# Autodesk Inventor assembly: Assembly1
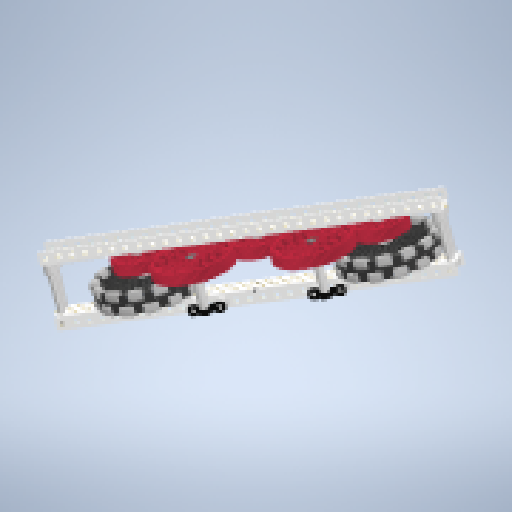
[picture p0: Inventor's stored thumbnail of the model, 512x512]
Saved by Autodesk Inventor 2024 (Build 280153000, 153)
## iProperties
Created: 2023-09-19
Part Number: Assembly1
Document SubType Name: Assembly
Designer: Robodox
Author: Robodox
## Documents named in this file (18)
- C:\Users\Robodox\Documents\GitHub\VEXCAD\Assembly1.iam
- C:\Users\Robodox\Documents\GitHub\VEX-CAD-Inventor\Structure\C Channel\Aluminum 1x2x1\Alu C 1x2x1x30.ipt
- C:\Users\Robodox\Documents\GitHub\VEX-CAD-Inventor\Motion\Gears\HS Gear.iam
- C:\Users\Robodox\Documents\GitHub\VEXCAD\Part1.ipt
- C:\Users\Robodox\Documents\GitHub\VEXCAD\Part2.ipt
- C:\Users\Robodox\Documents\GitHub\VEXCAD\Part3.ipt
- C:\Users\Robodox\Documents\GitHub\VEX-CAD-Inventor\Motion\Spacers\Washer Steel\SWasher .375 OD x .031250.ipt
- C:\Users\Robodox\Documents\GitHub\VEX-CAD-Inventor\Motion\Spacers\Washer Steel.ipt
- C:\Users\Robodox\Documents\GitHub\VEXCAD\Part4.ipt
- C:\Users\Robodox\Downloads\2020 VRC Library-BNS-SID-YY-EZ\2020 BNS-VRC-SID-YY Library\Motion\Pillow Bearing Block.ipt
- C:\Users\Robodox\Documents\GitHub\VEXCAD\Part5.ipt
- C:\Users\Robodox\Downloads\2020 VRC Library-BNS-SID-YY-EZ\2020 BNS-VRC-SID-YY Library\Motion\Bearing Flat.ipt
- C:\Users\Robodox\Documents\GitHub\VEXCAD\part8.ipt
- C:\Users\Robodox\Downloads\2020 VRC Library-BNS-SID-YY-EZ\2020 BNS-VRC-SID-YY Library\Motion\Shaft Collar.ipt
- C:\Users\Robodox\Documents\GitHub\VEX-CAD-Inventor\Motion\Wheels\Omni Wheel\4 Omni AS, Square.iam
- C:\Users\Robodox\Documents\GitHub\VEX-CAD-Inventor\Motion\Wheels\Omni Wheel.iam
- C:\Users\Robodox\Documents\GitHub\VEX-CAD-Inventor\Motion\Gears\HS Gear\HS 72T Gear, Square.iam
- C:\Users\Robodox\Documents\GitHub\VEX-CAD-Inventor\Motion\Gears\HS Gear\HS 48T Gear, Square.iam
## Components (61 placed, 14 different names)
1. Alu C 1x2x1x30:1 — Flush:1, Flush:2, Mate:1, Mate:2, Mate:7, Mate:11, Mate:12, Mate:15, Mate:17, Mate:19, Mate:27, Mate:31, Mate:32, Mate:33, Mate:34, Mate:35, Mate:36, Mate:37, Mate:38, Mate:56, Mate:57, Mate:58, Mate:59, Mate:60, Mate:61, Mate:62, Mate:63, Mate:64
2. Alu C 1x2x1x30:2 — Flush:1, Flush:2, Mate:20, Mate:21, Mate:68, Mate:71, Mate:74
3. Part2:5 — Mate:13, Mate:14, Mate:28, Mate:29
4. Part1:9 — Mate:14, Mate:29
5. Part1:10 — Mate:12, Mate:13, Mate:15, Mate:28
6. Part3:3 — Mate:31, Mate:32, Mate:39, Mate:40
7. Part3:4 — Mate:33, Mate:38, Mate:41
8. Part3:5 — Mate:34, Mate:37, Mate:42, Mate:43
9. Part3:6 — Mate:35, Mate:36, Mate:44
10. Pillow Bearing Block:1 — Mate:39, Mate:40, Mate:41, Mate:50, Mate:51
11. Pillow Bearing Block:2 — Mate:42, Mate:43, Mate:44, Mate:46, Mate:53
12. Part5:1 — Mate:47, Mate:52, Mate:94, Mate:96
13. Part5:2 — Mate:48, Mate:49, Mate:95, Mate:97
14. Part5:3 — Mate:46, Mate:47, Mate:52, Mate:53
15. Part5:4 — Mate:48, Mate:49, Mate:50, Mate:51
16. Bearing Flat:1 — Mate:56, Mate:59, Mate:60, Mate:72, Mate:86, Mate:88
17. Bearing Flat:2 — Mate:57, Mate:61, Mate:62, Mate:75
18. Bearing Flat:3 — Mate:58, Mate:63, Mate:64, Mate:69, Mate:91
19. part8:1 — Mate:68, Mate:69, Mate:98, Mate:99
20. part8:2 — Mate:71, Mate:72, Mate:106, Mate:107
21. part8:3 — Mate:74, Mate:75, Mate:102, Mate:103
22. Part3:11 — Mate:90
23. Part3:12 — Mate:87, Mate:100, Mate:101
24. Shaft Collar:1 — Mate:86, Mate:89, Mate:104, Mate:105
25. Shaft Collar:2 — Mate:92, Mate:93
26. 4 Omni AS, Square:1 [sub-assembly] — Mate:87, Mate:88, Mate:89
27. 4 Omni AS, Square:2 [sub-assembly] — Mate:90, Mate:91, Mate:92, Mate:93
28. HS 72T Gear, Square:8 [sub-assembly] — Mate:94, Mate:96
29. HS 72T Gear, Square:9 [sub-assembly] — Mate:95, Mate:97
30. HS 48T Gear, Square:10 [sub-assembly] — Mate:98, Mate:99
31. HS 48T Gear, Square:11 [sub-assembly] — Mate:100, Mate:101, Mate:106, Mate:107
32. HS 48T Gear, Square:12 [sub-assembly] — Mate:102, Mate:103
33. SWasher .375 OD x .031250:5 — Mate:104, Mate:105
34. Part1:1 — Mate:4, Mate:5
35. Part2:1 — Mate:3, Mate:4, Mate:5, Mate:6
36. Part1:2 — Mate:1, Mate:2, Mate:3, Mate:6
37. Part1:3
38. Part2:2
39. Part1:4
40. Part1:6 — Mate:9, Mate:10
41. Part2:3 — Mate:8, Mate:9, Mate:10, Mate:30
42. Part1:5 — Mate:7, Mate:8, Mate:11, Mate:30
43. Part1:7
44. Part2:4
45. Part1:8
46. Part1:11 — Mate:16, Mate:17, Mate:18, Mate:19, Mate:26
47. Part2:6 — Mate:16, Mate:18
48. Part1:12
49. Part2:7
50. Part3:1 — Mate:20, Mate:21, Mate:22, Mate:23, Mate:25
51. Part4:1 — Mate:24, Mate:25, Mate:26, Mate:27
52. SWasher .375 OD x .031250:1 — Mate:22, Mate:23, Mate:24
53. Part3:2
54. Part4:2
55. SWasher .375 OD x .031250:2
56. Part3:8
57. Part4:3
58. SWasher .375 OD x .031250:3
59. Part3:9
60. Part4:4
61. SWasher .375 OD x .031250:4
## Component patterns: (2 elements, first: Part1:1 + Part2:1 + Part1:2), (2 elements, first: Part1:6 + Part2:3 + Part1:5), (2 elements, first: Part1:11 + Part2:6), (2 elements), (2 elements, first: Part3:1 + Part4:1 + SWasher .375 OD x .031250:1), Component Pattern 4:2 (2 elements)
## Relationships (91: Mate 89, Flush 2)
- Flush:1: Alu C 1x2x1x30:1 ↔ Alu C 1x2x1x30:2
- Flush:2: Alu C 1x2x1x30:1 ↔ Alu C 1x2x1x30:2
- Mate:1: Alu C 1x2x1x30:1 ↔ Part1:2
- Mate:2: Alu C 1x2x1x30:1 ↔ Part1:2
- Mate:3: Part2:1 ↔ Part1:2
- Mate:4: Part1:1 ↔ Part2:1
- Mate:5: Part1:1 ↔ Part2:1
- Mate:6: Part2:1 ↔ Part1:2
- Mate:7: Alu C 1x2x1x30:1 ↔ Part1:5
- Mate:8: Part2:3 ↔ Part1:5
- Mate:9: Part1:6 ↔ Part2:3
- Mate:10: Part1:6 ↔ Part2:3
- Mate:11: Alu C 1x2x1x30:1 ↔ Part1:5
- Mate:12: Alu C 1x2x1x30:1 ↔ Part1:10
- Mate:13: Part2:5 ↔ Part1:10
- Mate:14: Part2:5 ↔ Part1:9
- Mate:15: Alu C 1x2x1x30:1 ↔ Part1:10
- Mate:16: Part1:11 ↔ Part2:6
- Mate:17: Alu C 1x2x1x30:1 ↔ Part1:11
- Mate:18: Part1:11 ↔ Part2:6
- Mate:19: Alu C 1x2x1x30:1 ↔ Part1:11
- Mate:20: Alu C 1x2x1x30:2 ↔ Part3:1
- Mate:21: Alu C 1x2x1x30:2 ↔ Part3:1
- Mate:22: Part3:1 ↔ SWasher .375 OD x .031250:1
- Mate:23: Part3:1 ↔ SWasher .375 OD x .031250:1
- Mate:24: Part4:1 ↔ SWasher .375 OD x .031250:1
- Mate:25: Part3:1 ↔ Part4:1
- Mate:26: Part1:11 ↔ Part4:1
- Mate:27: Alu C 1x2x1x30:1 ↔ Part4:1
- Mate:28: Part2:5 ↔ Part1:10
- Mate:29: Part2:5 ↔ Part1:9
- Mate:30: Part2:3 ↔ Part1:5
- Mate:31: Alu C 1x2x1x30:1 ↔ Part3:3
- Mate:32: Alu C 1x2x1x30:1 ↔ Part3:3
- Mate:33: Alu C 1x2x1x30:1 ↔ Part3:4
- Mate:34: Alu C 1x2x1x30:1 ↔ Part3:5
- Mate:35: Alu C 1x2x1x30:1 ↔ Part3:6
- Mate:36: Alu C 1x2x1x30:1 ↔ Part3:6
- Mate:37: Alu C 1x2x1x30:1 ↔ Part3:5
- Mate:38: Alu C 1x2x1x30:1 ↔ Part3:4
- Mate:39: Part3:3 ↔ Pillow Bearing Block:1
- Mate:40: Part3:3 ↔ Pillow Bearing Block:1
- Mate:41: Part3:4 ↔ Pillow Bearing Block:1
- Mate:42: Part3:5 ↔ Pillow Bearing Block:2
- Mate:43: Part3:5 ↔ Pillow Bearing Block:2
- Mate:44: Part3:6 ↔ Pillow Bearing Block:2
- Mate:46: Pillow Bearing Block:2 ↔ Part5:3
- Mate:47: Part5:1 ↔ Part5:3
- Mate:48: Part5:2 ↔ Part5:4
- Mate:49: Part5:2 ↔ Part5:4
- Mate:50: Pillow Bearing Block:1 ↔ Part5:4
- Mate:51: Pillow Bearing Block:1 ↔ Part5:4
- Mate:52: Part5:1 ↔ Part5:3
- Mate:53: Pillow Bearing Block:2 ↔ Part5:3
- Mate:56: Alu C 1x2x1x30:1 ↔ Bearing Flat:1
- Mate:57: Alu C 1x2x1x30:1 ↔ Bearing Flat:2
- Mate:58: Alu C 1x2x1x30:1 ↔ Bearing Flat:3
- Mate:59: Alu C 1x2x1x30:1 ↔ Bearing Flat:1
- Mate:60: Alu C 1x2x1x30:1 ↔ Bearing Flat:1
- Mate:61: Alu C 1x2x1x30:1 ↔ Bearing Flat:2
- Mate:62: Alu C 1x2x1x30:1 ↔ Bearing Flat:2
- Mate:63: Alu C 1x2x1x30:1 ↔ Bearing Flat:3
- Mate:64: Alu C 1x2x1x30:1 ↔ Bearing Flat:3
- Mate:68: Alu C 1x2x1x30:2 ↔ part8:1
- Mate:69: Bearing Flat:3 ↔ part8:1
- Mate:71: Alu C 1x2x1x30:2 ↔ part8:2
- Mate:72: Bearing Flat:1 ↔ part8:2
- Mate:74: Alu C 1x2x1x30:2 ↔ part8:3
- Mate:75: Bearing Flat:2 ↔ part8:3
- Mate:86: Bearing Flat:1 ↔ Shaft Collar:1
- Mate:87: Part3:12 ↔ 4 Omni AS, Square:1
- Mate:88: Bearing Flat:1 ↔ 4 Omni AS, Square:1
- Mate:89: Shaft Collar:1 ↔ 4 Omni AS, Square:1
- Mate:90: Part3:11 ↔ 4 Omni AS, Square:2
- Mate:91: Bearing Flat:3 ↔ 4 Omni AS, Square:2
- Mate:92: Shaft Collar:2 ↔ 4 Omni AS, Square:2
- Mate:93: Shaft Collar:2 ↔ 4 Omni AS, Square:2
- Mate:94: Part5:1 ↔ HS 72T Gear, Square:8
- Mate:95: Part5:2 ↔ HS 72T Gear, Square:9
- Mate:96: Part5:1 ↔ HS 72T Gear, Square:8
- Mate:97: Part5:2 ↔ HS 72T Gear, Square:9
- Mate:98: part8:1 ↔ HS 48T Gear, Square:10
- Mate:99: part8:1 ↔ HS 48T Gear, Square:10
- Mate:100: Part3:12 ↔ HS 48T Gear, Square:11
- Mate:101: Part3:12 ↔ HS 48T Gear, Square:11
- Mate:102: part8:3 ↔ HS 48T Gear, Square:12
- Mate:103: part8:3 ↔ HS 48T Gear, Square:12
- Mate:104: Shaft Collar:1 ↔ SWasher .375 OD x .031250:5
- Mate:105: Shaft Collar:1 ↔ SWasher .375 OD x .031250:5
- Mate:106: part8:2 ↔ HS 48T Gear, Square:11
- Mate:107: part8:2 ↔ HS 48T Gear, Square:11
